# Autodesk Inventor assembly: Link_5
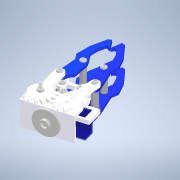
[picture p0: Inventor's stored thumbnail of the model, 180x180]
Saved by Autodesk Inventor 2022 (Build 260153000, 153)
## iProperties
Created: 2021-09-23
Part Number: Link_5
Document SubType Name: Assembly
Designer: Administrador
Author: Administrador
## Documents named in this file (3)
- C:\Users\Administrador\Desktop\Octavo Semestre\Robótica Industrial\Robot\Links\Link_5.iam
- C:\Users\Administrador\Desktop\Octavo Semestre\Robótica Industrial\Robot\Pinza\Ensamble Pinza.iam
- C:\Users\Administrador\Desktop\Octavo Semestre\Robótica Industrial\Robot\Cuerpo\PartesCuerpo\Estella Servo1.ipt
## Components (2 placed, 2 different names)
1. Ensamble Pinza:1 [sub-assembly]
2. Estella Servo1:1
## Relationships (2: Mate 1, WeldJoint 1)
- [Mate]: Ensamble Pinza:1 ↔ Estella Servo1:1
- [WeldJoint]: Ensamble Pinza:1 ↔ Estella Servo1:1
